# Autodesk Inventor assembly: !arm
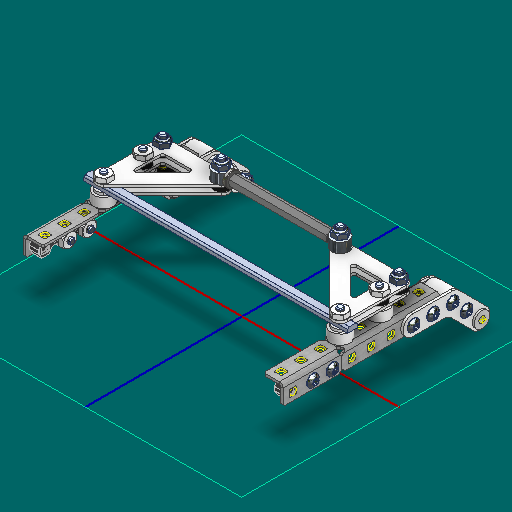
[picture p0: Inventor's stored thumbnail of the model, 512x512]
Saved by Autodesk Inventor 2025 (Build 290162000, 162)
## iProperties
Created: 2024-08-18
Part Number: !arm
Document SubType Name: Assembly
Designer: averey
Author: averey
## Documents named in this file (22)
- C:\Users\avere\vex_robotics_high_stakes\hardware\cad\ATLAS\intake\first_stage\arm\!arm.iam
- C:\Users\avere\vex_robotics_high_stakes\hardware\cad\ATLAS\intake\first_stage\arm\arm_half.iam
- C:\Users\avere\vex_robotics_high_stakes\hardware\cad\ATLAS\intake\first_stage\arm\arm_half_mirrored\arm_half_mirrored.iam
- C:\Users\avere\vex_robotics_high_stakes\hardware\cad\ATLAS\intake\first_stage\arm\custom_parts\hs_brace.ipt
- C:\Users\avere\vex_robotics_high_stakes\hardware\cad\ATLAS\chassis\structure\custom_parts\right_angle_gusset.ipt
- C:\Users\avere\vex_robotics_high_stakes\hardware\cad\VEX-CAD-Inventor\Motion\Spacers\Spacer Nylon .375 OD\NSpacer .375 OD x .125.ipt
- C:\Users\avere\vex_robotics_high_stakes\hardware\cad\VEX-CAD-Inventor\Motion\Spacers\Spacer Nylon .375 OD.ipt
- C:\Users\avere\vex_robotics_high_stakes\hardware\cad\VEX-CAD-Inventor\Motion\Shaft LS\Shaft Collar ipts\Shaft Collar No Screw.ipt
- C:\Users\avere\vex_robotics_high_stakes\hardware\cad\VEX-CAD-Inventor\Structure\Standoff\Standoff 2.50.ipt
- C:\Users\avere\vex_robotics_high_stakes\hardware\cad\VEX-CAD-Inventor\Structure\Standoff.ipt
- C:\Users\avere\vex_robotics_high_stakes\hardware\cad\VEX-CAD-Inventor\Motion\Spacers\Washer Steel.ipt
- C:\Users\avere\vex_robotics_high_stakes\hardware\cad\VEX-CAD-Inventor\Motion\Spacers\Washer Steel\SWasher .375 OD x .031250.ipt
- C:\Users\avere\vex_robotics_high_stakes\hardware\cad\VEX-CAD-Inventor\Motion\Spacers\Washer Steel\SWasher .375 OD x .062500.ipt
- C:\Users\avere\vex_robotics_high_stakes\hardware\cad\VEX-CAD-Inventor\Structure\Hardware\Screw Steel - Star\SScrew Star Smooth .750.ipt
- C:\Users\avere\vex_robotics_high_stakes\hardware\cad\VEX-CAD-Inventor\Structure\Hardware\Screw Steel - Star.ipt
- C:\Users\avere\vex_robotics_high_stakes\hardware\cad\VEX-CAD-Inventor\Structure\Hardware\Nut Thin Nylock.ipt
- C:\Users\avere\vex_robotics_high_stakes\hardware\cad\VEX-CAD-Inventor\Motion\Spacers\Spacer Nylon .500 OD\NSpacer White .500 OD x .250.ipt
- C:\Users\avere\vex_robotics_high_stakes\hardware\cad\VEX-CAD-Inventor\Motion\Spacers\Spacer Nylon .500 OD.ipt
- C:\Users\avere\vex_robotics_high_stakes\hardware\cad\VEX-CAD-Inventor\Structure\Hardware\Screw Shoulder Robosource\SScrew Shoulder Smooth .500 x .04.ipt
- C:\Users\avere\vex_robotics_high_stakes\hardware\cad\VEX-CAD-Inventor\Structure\Hardware\Screw Shoulder Robosource.ipt
- C:\Users\avere\vex_robotics_high_stakes\hardware\cad\VEX-CAD-Inventor\Structure\Hardware\Nut Nylon\Nut Nylon - White.ipt
- C:\Users\avere\vex_robotics_high_stakes\hardware\cad\VEX-CAD-Inventor\Structure\Hardware\Nut Nylon.ipt
## Components (38 placed, 14 different names)
1. arm_half:1 [sub-assembly] — Mate:1, Mate:2, Insert:1, Mate:5, Insert:26, Insert:27, Insert:38, Insert:39
2. arm_half_mirrored:1 [sub-assembly] — Mate:4, Insert:1, Mate:5, Insert:13, Mate:8, Insert:24, Insert:25, Insert:32, Insert:33
3. hs_brace:1 — Insert:2, Insert:3, Insert:12
4. right_angle_gusset:1 — Insert:3, Mate:6, Insert:7, Insert:13, Mate:8, Insert:20, Insert:28
5. right_angle_gusset:2 — Insert:2, Mate:6, Insert:4, Insert:5, Insert:6, Flush:1, Insert:14, Insert:34, Insert:35
6. NSpacer .375 OD x .125:1 — Insert:4
7. NSpacer .375 OD x .125:2 — Insert:5
8. NSpacer .375 OD x .125:3 — Insert:6, Insert:7
9. right_angle_gusset:3 — Flush:1, Insert:15, Insert:36, Insert:37
10. right_angle_gusset:4 — Insert:12, Insert:21, Insert:31
11. NSpacer .375 OD x .125:4
12. NSpacer .375 OD x .125:5
13. NSpacer .375 OD x .125:6
14. Shaft Collar No Screw:1 — Insert:14, Mate:9, Insert:19, Insert:22
15. Shaft Collar No Screw:2 — Insert:15, Mate:9, Insert:23
16. Standoff 2.50:1 — Insert:17
17. SWasher .375 OD x .031250:2 — Insert:17, Insert:18
18. SWasher .375 OD x .062500:3 — Insert:18, Insert:19
19. SScrew Star Smooth .750:1 — Insert:20
20. SScrew Star Smooth .750:2 — Insert:21
21. Nut Thin Nylock:1 — Insert:23
22. Nut Thin Nylock:2 — Insert:22
23. NSpacer White .500 OD x .250:1 — Insert:24
24. NSpacer White .500 OD x .250:2 — Insert:25
25. NSpacer White .500 OD x .250:3 — Insert:26
26. NSpacer White .500 OD x .250:4 — Insert:27
27. SScrew Shoulder Smooth .500 x .04:1 — Insert:28, Insert:29
28. Nut Thin Nylock:3 — Insert:29
29. SScrew Shoulder Smooth .500 x .04:2 — Insert:31
30. Nut Thin Nylock:4
31. SScrew Star Smooth .750:3 — Insert:32
32. SScrew Star Smooth .750:4 — Insert:33
33. Nut Nylon - White:1 — Insert:34
34. Nut Nylon - White:2 — Insert:35
35. Nut Nylon - White:3 — Insert:37
36. Nut Nylon - White:4 — Insert:36
37. SScrew Star Smooth .750:5 — Insert:39
38. SScrew Star Smooth .750:6 — Insert:38
## Relationships (47: Insert 38, Mate 8, Flush 1)
- Mate:1 (5.9309 mm): arm_half:1
- Mate:2 (82.4706 mm): arm_half:1
- Mate:4 (5.9309 mm): arm_half_mirrored:1
- Insert:1 (164.9412 mm): arm_half:1 ↔ arm_half_mirrored:1
- Mate:5: arm_half:1 ↔ arm_half_mirrored:1
- Insert:2: hs_brace:1 ↔ right_angle_gusset:2
- Insert:3: hs_brace:1 ↔ right_angle_gusset:1
- Mate:6: right_angle_gusset:1 ↔ right_angle_gusset:2
- Insert:4: right_angle_gusset:2 ↔ NSpacer .375 OD x .125:1
- Insert:5: right_angle_gusset:2 ↔ NSpacer .375 OD x .125:2
- Insert:6: right_angle_gusset:2 ↔ NSpacer .375 OD x .125:3
- Insert:7: right_angle_gusset:1 ↔ NSpacer .375 OD x .125:3
- [Mate]: right_angle_gusset:3 ↔ right_angle_gusset:4
- [Insert]: right_angle_gusset:4 ↔ NSpacer .375 OD x .125:4
- [Insert]: right_angle_gusset:4 ↔ NSpacer .375 OD x .125:5
- [Insert]: right_angle_gusset:4 ↔ NSpacer .375 OD x .125:6
- [Insert]: right_angle_gusset:3 ↔ NSpacer .375 OD x .125:6
- Insert:12: hs_brace:1 ↔ right_angle_gusset:4
- Flush:1: right_angle_gusset:2 ↔ right_angle_gusset:3
- Insert:13 (6.35 mm): arm_half_mirrored:1 ↔ right_angle_gusset:1
- Mate:8: arm_half_mirrored:1 ↔ right_angle_gusset:1
- Insert:14: right_angle_gusset:2 ↔ Shaft Collar No Screw:1
- Insert:15: right_angle_gusset:3 ↔ Shaft Collar No Screw:2
- Mate:9: Shaft Collar No Screw:1 ↔ Shaft Collar No Screw:2
- Insert:17: Standoff 2.50:1 ↔ SWasher .375 OD x .031250:2
- Insert:18: SWasher .375 OD x .031250:2 ↔ SWasher .375 OD x .062500:3
- Insert:19: Shaft Collar No Screw:1 ↔ SWasher .375 OD x .062500:3
- Insert:20: right_angle_gusset:1 ↔ SScrew Star Smooth .750:1
- Insert:21: right_angle_gusset:4 ↔ SScrew Star Smooth .750:2
- Insert:22: Shaft Collar No Screw:1 ↔ Nut Thin Nylock:2
- Insert:23: Shaft Collar No Screw:2 ↔ Nut Thin Nylock:1
- Insert:24: arm_half_mirrored:1 ↔ NSpacer White .500 OD x .250:1
- Insert:25: arm_half_mirrored:1 ↔ NSpacer White .500 OD x .250:2
- Insert:26: arm_half:1 ↔ NSpacer White .500 OD x .250:3
- Insert:27: arm_half:1 ↔ NSpacer White .500 OD x .250:4
- Insert:28: right_angle_gusset:1 ↔ SScrew Shoulder Smooth .500 x .04:1
- Insert:29 (6.35 mm): SScrew Shoulder Smooth .500 x .04:1 ↔ Nut Thin Nylock:3
- [Insert] (6.35 mm): SScrew Shoulder Smooth .500 x .04:2 ↔ Nut Thin Nylock:4
- Insert:31: right_angle_gusset:4 ↔ SScrew Shoulder Smooth .500 x .04:2
- Insert:32: arm_half_mirrored:1 ↔ SScrew Star Smooth .750:3
- Insert:33: arm_half_mirrored:1 ↔ SScrew Star Smooth .750:4
- Insert:34: right_angle_gusset:2 ↔ Nut Nylon - White:1
- Insert:35: right_angle_gusset:2 ↔ Nut Nylon - White:2
- Insert:36: right_angle_gusset:3 ↔ Nut Nylon - White:4
- Insert:37: right_angle_gusset:3 ↔ Nut Nylon - White:3
- Insert:38: arm_half:1 ↔ SScrew Star Smooth .750:6
- Insert:39: arm_half:1 ↔ SScrew Star Smooth .750:5
## Named parameters: d19_d13 = 0 mm, d20_d15 = 0 mm, d21_d16 = 0 mm, d22_d17 = 0 mm, d23_d18 = 0 mm, d46_d45 = 6.35 mm
